# Autodesk Inventor assembly: Assembly_XY_stage_with_motors_v3
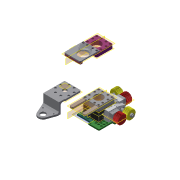
[picture p0: Inventor's stored thumbnail of the model, 180x180]
Saved by Autodesk Inventor 2022 (Build 260153000, 153)
## iProperties
Created: 2021-02-08
Part Number: Assembly_XY_stage_with_motors_v3
Document SubType Name: Assembly
Designer: diederichbenedict
Author: diederichbenedict
## Documents named in this file (10)
- C:\Users\diederichbenedict\Dropbox\Dokumente\Promotion\PROJECTS\UC2\02_CAD\INVENTOR\uc2_v3\Assembly_XY_stage_with_motors_v3.iam
- C:\Users\diederichbenedict\Dropbox\Dokumente\Promotion\PROJECTS\UC2\02_CAD\INVENTOR\uc2_v3\00_XY_stage-CHUO_SEIKI_LD-647-R1.iam
- C:\Users\diederichbenedict\Dropbox\Dokumente\Promotion\PROJECTS\UC2\02_CAD\INVENTOR\uc2_v3\30_XY_Sample_arm_v3.ipt
- C:\Users\diederichbenedict\Dropbox\Dokumente\Promotion\PROJECTS\UC2\02_CAD\INVENTOR\uc2_v3\30_cellSTORM_UC2_Laser_base.ipt
- C:\Users\diederichbenedict\Dropbox\Dokumente\Promotion\PROJECTS\UC2\02_CAD\INVENTOR\uc2_v3\30_cellSTORM_UC2_motorized_xystage_spacer.ipt
- C:\Users\diederichbenedict\Dropbox\Dokumente\Promotion\PROJECTS\UC2\02_CAD\INVENTOR\uc2_v3\30_cellSTORM_UC2_Sample_arm_ptycho.ipt
- C:\Users\diederichbenedict\Dropbox\Dokumente\Promotion\PROJECTS\UC2\02_CAD\INVENTOR\uc2_v3\Assembly_Nema_Motor_attachement_for_XYstage.iam
- C:\Users\diederichbenedict\Dropbox\Dokumente\Promotion\PROJECTS\UC2\02_CAD\INVENTOR\uc2_v3\00_SMLM_chamber.ipt
- C:\Users\diederichbenedict\Dropbox\Dokumente\Promotion\PROJECTS\UC2\02_CAD\INVENTOR\uc2_v3\30_cellSTORM_XY_Sample_arm_90degRot_v3.ipt
- C:\Users\diederichbenedict\Dropbox\Dokumente\Promotion\PROJECTS\UC2\02_CAD\INVENTOR\uc2_v3\30_cellSTORM_XY_Sample_arm_35mmadapter.ipt
## Components (10 placed, 9 different names)
1. 00_XY_stage-CHUO_SEIKI_LD-647-R1:1 [sub-assembly] — Insert:2, Mate:3, Einfügen:3
2. 30_XY_Sample_arm_v3:1 — Flush:1
3. 30_cellSTORM_UC2_Laser_base:1 — Insert:2, Flush:3
4. 30_cellSTORM_UC2_motorized_xystage_spacer:1 — Flush:1
5. 30_cellSTORM_UC2_Sample_arm_ptycho:1
6. Assembly_Nema_Motor_attachement_for_XYstage:1 [sub-assembly] — Mate:3, Flush:3
7. 00_SMLM_chamber:1 — Tangent:1, Mate:5, Tangent:2
8. 30_cellSTORM_XY_Sample_arm_90degRot_v3:1 — Tangent:1, Mate:5, Tangent:2, Flush:4, Flush:5
9. 30_cellSTORM_XY_Sample_arm_35mmadapter:1 — Flush:4, Flush:5
10. Assembly_Nema_Motor_attachement_for_XYstage:2 [sub-assembly] — Einfügen:3
## Relationships (12: Flush 4, Insert 3, Mate 2, Tangent 2, Angle 1)
- [Insert]: 00_XY_stage-CHUO_SEIKI_LD-647-R1:1 ↔ 30_XY_Sample_arm_v3:1
- [Angle] (0 deg): 00_XY_stage-CHUO_SEIKI_LD-647-R1:1 ↔ 30_cellSTORM_UC2_Laser_base:1
- Insert:2: 00_XY_stage-CHUO_SEIKI_LD-647-R1:1 ↔ 30_cellSTORM_UC2_Laser_base:1
- Flush:1: 30_XY_Sample_arm_v3:1 ↔ 30_cellSTORM_UC2_motorized_xystage_spacer:1
- Mate:3: 00_XY_stage-CHUO_SEIKI_LD-647-R1:1 ↔ Assembly_Nema_Motor_attachement_for_XYstage:1
- Flush:3 (10 mm): 30_cellSTORM_UC2_Laser_base:1 ↔ Assembly_Nema_Motor_attachement_for_XYstage:1
- Tangent:1 (10 mm): 00_SMLM_chamber:1 ↔ 30_cellSTORM_XY_Sample_arm_90degRot_v3:1
- Mate:5 (5 mm): 00_SMLM_chamber:1 ↔ 30_cellSTORM_XY_Sample_arm_90degRot_v3:1
- Tangent:2 (10 mm): 00_SMLM_chamber:1 ↔ 30_cellSTORM_XY_Sample_arm_90degRot_v3:1
- Flush:4: 30_cellSTORM_XY_Sample_arm_90degRot_v3:1 ↔ 30_cellSTORM_XY_Sample_arm_35mmadapter:1
- Flush:5: 30_cellSTORM_XY_Sample_arm_90degRot_v3:1 ↔ 30_cellSTORM_XY_Sample_arm_35mmadapter:1
- Einfügen:3 [Insert]: 00_XY_stage-CHUO_SEIKI_LD-647-R1:1 ↔ Assembly_Nema_Motor_attachement_for_XYstage:2
